# Autodesk Inventor assembly: AutotunerCAD
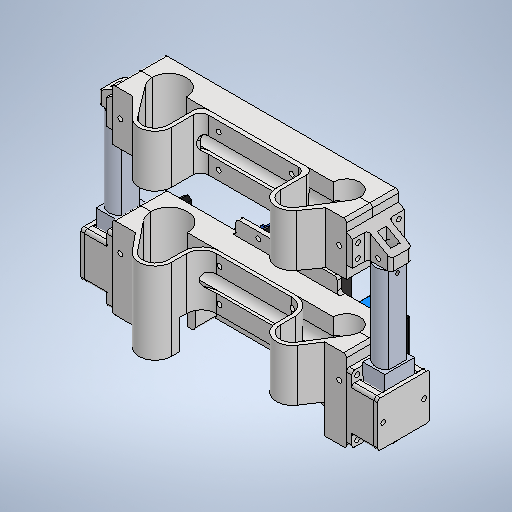
[picture p0: Inventor's stored thumbnail of the model, 512x512]
Saved by Autodesk Inventor 2026 (Build 300175050, 175E)
## iProperties
Created: 2025-12-10
Part Number: AutotunerCAD
Document SubType Name: Assembly
Designer: Nicholas M
Author: Nicholas M
## Documents named in this file (13)
- C:\Users\nmari\OneDrive\Desktop\Trombone-Autotuner\AutotunerCAD.iam
- C:\Users\nmari\OneDrive\Desktop\Trombone-Autotuner\BottomHalf2.ipt
- C:\Users\nmari\OneDrive\Desktop\Trombone-Autotuner\BottomHalf1.ipt
- C:\Users\nmari\OneDrive\Desktop\Trombone-Autotuner\MotorMount.ipt
- C:\Users\nmari\OneDrive\Desktop\Trombone-Autotuner\FIT0805.ipt
- C:\Users\nmari\OneDrive\Desktop\Trombone-Autotuner\BottomMountTop.ipt
- C:\Users\nmari\OneDrive\Desktop\Trombone-Autotuner\M3Adapter.ipt
- C:\Users\nmari\OneDrive\Desktop\Trombone-Autotuner\TopMotorMount.ipt
- C:\Users\nmari\OneDrive\Desktop\Trombone-Autotuner\TopHalf1.ipt
- C:\Users\nmari\OneDrive\Desktop\Trombone-Autotuner\TopHalf2.ipt
- C:\Users\nmari\OneDrive\Desktop\Trombone-Autotuner\Arduino_Uno_Q_V0.ipt
- C:\Users\nmari\OneDrive\Desktop\Trombone-Autotuner\hexstandoff.ipt
- C:\Users\nmari\OneDrive\Desktop\Trombone-Autotuner\battery.ipt
## Components (24 placed, 12 different names)
1. BottomHalf1:1 — Mate:1, Mate:2, Flush:1, Mate:3, Mate:17, Mate:21, Mate:32, Mate:33, Mate:44, Mate:45, Rigid:1, Rigid:2
2. BottomHalf2:1 — Mate:1, Mate:2, Flush:1, Mate:16, Mate:19, Mate:20
3. MotorMount:1 — Mate:3, Mate:11, Mate:12, Angle:2, Mate:14, Mate:15, Mate:16, Mate:17, Mate:18
4. MotorMount:2 — Mate:9, Mate:10, Angle:1, Mate:19, Mate:20, Mate:21, Mate:22, Mate:23, Mate:24
5. FIT0805:1 — Mate:9, Mate:10, Angle:1, Mate:26, Flush:3, Angle:4, Mate:29, Mate:30, Mate:31
6. FIT0805:2 — Mate:11, Mate:12, Angle:2, Mate:25, Flush:2
7. BottomMountTop:1 — Mate:14, Mate:15, Mate:18
8. BottomMountTop:2 — Mate:22, Mate:23, Mate:24
9. M3Adapter:1 — Mate:25, Flush:2
10. M3Adapter:2 — Mate:26, Flush:3
11. TopMotorMount:1 — Mate:40, Mate:42, Mate:43
12. TopMotorMount:2 — Angle:4, Mate:29, Mate:30, Mate:31, Mate:34
13. TopHalf1:1 — Mate:32, Mate:33, Mate:34, Mate:35, Mate:41, Flush:4, Mate:43
14. TopHalf2:1 — Mate:35, Mate:40, Mate:41, Flush:4, Mate:42
15. Arduino_Uno_Q_V0:1 — Mate:44, Mate:45, Mate:46
16. battery:1 — Rigid:2
17. hexstandoff:1 — Rigid:1
18. hexstandoff:2
19. hexstandoff:3
20. hexstandoff:4
21. hexstandoff:5
22. hexstandoff:6
23. hexstandoff:7 — Mate:46
24. hexstandoff:8
## Component patterns: (8 elements, first: hexstandoff:1)
## Relationships (43: Mate 34, Flush 4, Angle 3, WeldJoint 2)
- Mate:1: BottomHalf1:1 ↔ BottomHalf2:1
- Mate:2: BottomHalf1:1 ↔ BottomHalf2:1
- Flush:1: BottomHalf1:1 ↔ BottomHalf2:1
- Mate:3: BottomHalf1:1 ↔ MotorMount:1
- Mate:9: MotorMount:2 ↔ FIT0805:1
- Mate:10: MotorMount:2 ↔ FIT0805:1
- Angle:1 (180 deg): MotorMount:2 ↔ FIT0805:1
- Mate:11: MotorMount:1 ↔ FIT0805:2
- Mate:12: MotorMount:1 ↔ FIT0805:2
- Angle:2 (180 deg): MotorMount:1 ↔ FIT0805:2
- Mate:14: MotorMount:1 ↔ BottomMountTop:1
- Mate:15: MotorMount:1 ↔ BottomMountTop:1
- Mate:16: BottomHalf2:1 ↔ MotorMount:1
- Mate:17: BottomHalf1:1 ↔ MotorMount:1
- Mate:18: MotorMount:1 ↔ BottomMountTop:1
- Mate:19: BottomHalf2:1 ↔ MotorMount:2
- Mate:20: BottomHalf2:1 ↔ MotorMount:2
- Mate:21: BottomHalf1:1 ↔ MotorMount:2
- Mate:22: MotorMount:2 ↔ BottomMountTop:2
- Mate:23: MotorMount:2 ↔ BottomMountTop:2
- Mate:24: MotorMount:2 ↔ BottomMountTop:2
- Mate:25: FIT0805:2 ↔ M3Adapter:1
- Flush:2: FIT0805:2 ↔ M3Adapter:1
- Mate:26: FIT0805:1 ↔ M3Adapter:2
- Flush:3: FIT0805:1 ↔ M3Adapter:2
- Angle:4 (180 deg): FIT0805:1 ↔ TopMotorMount:2
- Mate:29 (0.5 mm): FIT0805:1 ↔ TopMotorMount:2
- Mate:30 (1.525 mm): FIT0805:1 ↔ TopMotorMount:2
- Mate:31 (3.125 mm): FIT0805:1 ↔ TopMotorMount:2
- Mate:32: BottomHalf1:1 ↔ TopHalf1:1
- Mate:33: BottomHalf1:1 ↔ TopHalf1:1
- Mate:34: TopMotorMount:2 ↔ TopHalf1:1
- Mate:35: TopHalf1:1 ↔ TopHalf2:1
- Mate:40: TopMotorMount:1 ↔ TopHalf2:1
- Mate:41: TopHalf1:1 ↔ TopHalf2:1
- Flush:4: TopHalf1:1 ↔ TopHalf2:1
- Mate:42: TopMotorMount:1 ↔ TopHalf2:1
- Mate:43: TopMotorMount:1 ↔ TopHalf1:1
- Mate:44: BottomHalf1:1 ↔ Arduino_Uno_Q_V0:1
- Mate:45: BottomHalf1:1 ↔ Arduino_Uno_Q_V0:1
- Rigid:1 [WeldJoint]: BottomHalf1:1 ↔ hexstandoff:1
- Mate:46: Arduino_Uno_Q_V0:1 ↔ hexstandoff:7
- Rigid:2 [WeldJoint]: BottomHalf1:1 ↔ battery:1
